# Autodesk Inventor assembly: x_motor
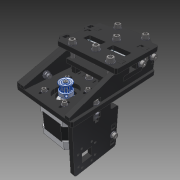
[picture p0: Inventor's stored thumbnail of the model, 180x180]
Saved by Autodesk Inventor 2014 (Build 180170000, 170)
## iProperties
Created: 2014-01-10
Part Number: x_motor
Document SubType Name: Assembly
Designer: buben
Author: buben
## Documents named in this file (23)
- C:\Users\buben\Documents\GitHub\bacon\inventor files\assemblies\x_motor.iam
- C:\Users\buben\Documents\GitHub\bacon\inventor files\printer parts\x_motor_back.ipt
- C:\Users\buben\Documents\GitHub\bacon\inventor files\printer parts\x_motor_wall_lower.ipt
- C:\Users\buben\Documents\GitHub\bacon\inventor files\printer parts\x_motor_wall_upper.ipt
- C:\Users\buben\Documents\GitHub\bacon\inventor files\printer parts\x_motor_middle.ipt
- C:\Users\buben\Documents\GitHub\bacon\inventor files\printer parts\x_motor_smooth_rod_spacer.ipt
- C:\Users\buben\Documents\GitHub\bacon\inventor files\3rd party components\linear_bearing_8\Imported Components\LU8MM\LU8MM.iam
- C:\Users\buben\Documents\GitHub\bacon\inventor files\printer parts\x_motor_top.ipt
- C:\Users\buben\Documents\GitHub\bacon\inventor files\printer parts\x_motor_upper_nut_stop.ipt
- C:\Users\buben\Documents\GitHub\bacon\inventor files\printer parts\x_motor_lower_nut_stop.ipt
- C:\Users\buben\Documents\GitHub\bacon\inventor files\utils\washer_m5.ipt
- C:\Users\buben\Documents\Inventor\Content Center Files\R2014\en-US\ISO 4762(2)\ISO 4762 - M5 x 45ISO.ipt
- C:\Users\buben\Documents\Inventor\Content Center Files\R2014\en-US\ISO 7040\ISO 7040 - M5.ipt
- C:\Users\buben\Documents\GitHub\bacon\inventor files\utils\washer_m4.ipt
- C:\Users\buben\Documents\Inventor\Content Center Files\R2014\en-US\ISO 4762(2)\ISO 4762 - M4 x 20ISO.ipt
- C:\Users\buben\Documents\Inventor\Content Center Files\R2014\en-US\ISO 7040\ISO 7040 - M4.ipt
- C:\Users\buben\Documents\GitHub\bacon\inventor files\printer parts\x_motor_cable_mount.ipt
- C:\Users\buben\Documents\GitHub\bacon\inventor files\printer parts\x_motor_cable_mount_brace.ipt
- C:\Users\buben\Documents\Inventor\Content Center Files\R2014\en-US\CSN EN 24032\ISO 4032 - M5CSN EN.ipt
- C:\Users\buben\Documents\GitHub\bacon\inventor files\printer parts\motor_spacer.ipt
- C:\Users\buben\Documents\GitHub\bacon\inventor files\3rd party components\nema_17_stepper\Imported Components\NEMA 17 with T5 Pulley\NEMA 17 with T5 Pulley.iam
- C:\Users\buben\Documents\GitHub\bacon\inventor files\utils\washer_m3.ipt
- C:\Users\buben\Documents\Inventor\Content Center Files\R2014\en-US\ISO 4762(2)\ISO 4762 - M3 x 16ISO.ipt
## Components (73 placed, 22 different names)
1. x_motor_back:1 — Mate:1, Flush:1, Mate:2, Mate:4, Mate:5, Mate:6, Mate:7, Mate:8, Mate:9, Mate:12, Mate:13, Mate:14, Mate:15, Mate:16, Mate:17, Mate:33, Mate:34, Mate:47, Mate:48, Mate:49, Mate:50, Mate:51, Mate:52, Mate:101, Mate:102, Mate:103, Mate:104, Mate:105, Mate:106, Mate:107, Mate:109, Mate:131, Tangent:1, Tangent:2, Mate:135, Mate:136, Mate:137, Mate:138
2. x_motor_wall_lower:1 — Mate:7, Mate:8, Mate:9, Mate:27, Mate:28, Mate:30, Mate:31, Mate:80, Mate:81, Mate:82, Mate:83, Mate:125, Mate:126
3. x_motor_wall_upper:1 — Mate:4, Mate:5, Mate:6, Mate:10, Mate:11, Mate:18, Mate:32, Mate:77, Mate:128, Mate:129
4. x_motor_middle:1 — Mate:10, Mate:11, Mate:18, Mate:19, Mate:20, Mate:21, Mate:22, Mate:23, Mate:24, Mate:29
5. x_motor_smooth_rod_spacer:1 — Mate:12, Mate:13, Mate:14
6. x_motor_smooth_rod_spacer:2 — Mate:15, Mate:16, Mate:17
7. LU8MM:1 [sub-assembly] — Mate:21, Mate:22, Mate:24
8. LU8MM:2 [sub-assembly] — Mate:19, Mate:20, Mate:23, Mate:25, Mate:26
9. x_motor_top:1 — Mate:25, Mate:26, Mate:27, Mate:28, Mate:35, Mate:36, Mate:37, Mate:38, Mate:39, Mate:40, Mate:41, Mate:42, Mate:43, Mate:44, Mate:45, Mate:46
10. x_motor_upper_nut_stop:1 — Mate:32, Mate:33, Mate:34, Mate:71, Mate:76, Mate:130
11. x_motor_lower_nut_stop:1 — Mate:29, Mate:30, Mate:31, Mate:84, Mate:85, Mate:127
12. CSN 02 1702 B B 5,3:1 — Mate:40, Mate:44, Insert:5
13. CSN 02 1702 B B 5,3:2 — Mate:38, Mate:42, Insert:2
14. CSN 02 1702 B B 5,3:3 — Mate:39, Mate:45, Insert:6
15. CSN 02 1702 B B 5,3:4 — Mate:37, Mate:46, Insert:3
16. CSN 02 1702 B B 5,3:5 — Mate:36, Mate:41, Insert:1
17. CSN 02 1702 B B 5,3:6 — Mate:35, Mate:43, Insert:4
18. CSN 02 1702 B B 5,3:7 — Mate:48, Mate:57, Mate:61
19. CSN 02 1702 B B 5,3:8 — Mate:51, Mate:54, Mate:63
20. CSN 02 1702 B B 5,3:9 — Mate:47, Mate:53, Mate:69
21. CSN 02 1702 B B 5,3:10 — Mate:49, Mate:56, Mate:65
22. CSN 02 1702 B B 5,3:11 — Mate:50, Mate:55, Mate:67
23. CSN 02 1702 B B 5,3:12 — Mate:52, Mate:58, Mate:59
24. ISO 4762 M5 x 45:1 — Insert:1, Mate:53, Mate:70
25. ISO 4762 M5 x 45:2 — Insert:2, Mate:54, Mate:64
26. ISO 4762 M5 x 45:3 — Insert:3, Mate:58, Mate:60
27. ISO 4762 M5 x 45:4 — Insert:4, Mate:56, Mate:66
28. ISO 4762 M5 x 45:5 — Insert:5, Mate:55, Mate:68
29. ISO 4762 M5 x 45:6 — Insert:6, Mate:57, Mate:62
30. DIN EN ISO 7040 M5:1 — Mate:69, Mate:70
31. DIN EN ISO 7040 M5:2 — Mate:67, Mate:68
32. DIN EN ISO 7040 M5:3 — Mate:65, Mate:66
33. DIN EN ISO 7040 M5:4 — Mate:63, Mate:64
34. DIN EN ISO 7040 M5:5 — Mate:61, Mate:62
35. DIN EN ISO 7040 M5:6 — Mate:59, Mate:60
36. CSN 02 1702 B B 4,3:2 — Mate:77, Mate:90, Mate:91
37. CSN 02 1702 B B 4,3:4 — Mate:71, Mate:76, Insert:7
38. CSN 02 1702 B B 4,3:7 — Mate:84, Mate:88, Mate:97
39. CSN 02 1702 B B 4,3:8 — Mate:85, Mate:89, Mate:99
40. CSN 02 1702 B B 4,3:9 — Mate:81, Mate:83, Insert:11
41. CSN 02 1702 B B 4,3:10 — Mate:80, Mate:82, Insert:10
42. ISO 4762 M4 x 20:1 — Insert:7, Mate:90, Mate:92
43. ISO 4762 M4 x 20:4 — Insert:10, Mate:89, Mate:100
44. ISO 4762 M4 x 20:5 — Insert:11, Mate:88, Mate:98
45. DIN EN ISO 7040 M4:3 — Mate:97, Mate:98
46. DIN EN ISO 7040 M4:4 — Mate:99, Mate:100
47. DIN EN ISO 7040 M4:5 — Mate:91, Mate:92
48. CSN 02 1702 B B 4,3:11 — Mate:101, Mate:102, Insert:12
49. CSN 02 1702 B B 4,3:12 — Mate:103, Mate:104, Insert:13
50. ISO 4762 M4 x 20:6 — Insert:12, Mate:118, Mate:124
51. ISO 4762 M4 x 20:7 — Insert:13, Mate:116, Mate:122
52. CSN 02 1702 B B 4,3:13 — Mate:115, Mate:116, Mate:121
53. CSN 02 1702 B B 4,3:14 — Mate:117, Mate:118, Mate:123
54. x_motor_cable_mount:1 — Mate:105, Mate:106, Mate:107, Mate:108, Mate:110, Mate:111, Mate:112, Mate:117
55. x_motor_cable_mount_brace:1 — Mate:108, Mate:109, Mate:110, Mate:113, Mate:115
56. CSN 02 1702 B B 4,3:15 — Mate:113, Mate:114, Mate:119
57. CSN 02 1702 B B 4,3:16 — Mate:111, Mate:112, Insert:14
58. ISO 4762 M4 x 20:8 — Insert:14, Mate:114, Mate:120
59. DIN EN ISO 7040 M4:6 — Mate:123, Mate:124
60. DIN EN ISO 7040 M4:7 — Mate:121, Mate:122
61. DIN EN ISO 7040 M4:8 — Mate:119, Mate:120
62. CSN EN 24032 M5:1 — Mate:128, Mate:129, Mate:130
63. CSN EN 24032 M5:2 — Mate:125, Mate:126, Mate:127
64. motor_spacer:1 — Mate:131, Tangent:1, Tangent:2, Mate:132, Mate:133, Mate:134, Mate:139, Mate:140, Mate:141, Mate:142
65. NEMA 17 with T5 Pulley:1 [sub-assembly] — Mate:132, Mate:133, Mate:134
66. CSN 02 1702 B B 3,2:1 — Mate:135, Insert:16
67. CSN 02 1702 B B 3,2:2 — Mate:136, Insert:15
68. CSN 02 1702 B B 3,2:3 — Mate:137, Insert:17
69. CSN 02 1702 B B 3,2:4 — Mate:138, Insert:18
70. ISO 4762 M3 x 16:1 — Insert:16, Mate:141
71. ISO 4762 M3 x 16:2 — Insert:15, Mate:139
72. ISO 4762 M3 x 16:3 — Insert:17, Mate:142
73. ISO 4762 M3 x 16:4 — Insert:18, Mate:140
## Relationships (148: Mate 129, Insert 16, Tangent 2, Flush 1)
- Mate:1: x_motor_back:1
- Flush:1: x_motor_back:1
- Mate:2: x_motor_back:1
- Mate:4: x_motor_back:1 ↔ x_motor_wall_upper:1
- Mate:5: x_motor_back:1 ↔ x_motor_wall_upper:1
- Mate:6: x_motor_back:1 ↔ x_motor_wall_upper:1
- Mate:7: x_motor_back:1 ↔ x_motor_wall_lower:1
- Mate:8: x_motor_back:1 ↔ x_motor_wall_lower:1
- Mate:9: x_motor_back:1 ↔ x_motor_wall_lower:1
- Mate:10: x_motor_wall_upper:1 ↔ x_motor_middle:1
- Mate:11: x_motor_wall_upper:1 ↔ x_motor_middle:1
- Mate:12: x_motor_back:1 ↔ x_motor_smooth_rod_spacer:1
- Mate:13: x_motor_back:1 ↔ x_motor_smooth_rod_spacer:1
- Mate:14: x_motor_back:1 ↔ x_motor_smooth_rod_spacer:1
- Mate:15: x_motor_back:1 ↔ x_motor_smooth_rod_spacer:2
- Mate:16: x_motor_back:1 ↔ x_motor_smooth_rod_spacer:2
- Mate:17: x_motor_back:1 ↔ x_motor_smooth_rod_spacer:2
- Mate:18: x_motor_wall_upper:1 ↔ x_motor_middle:1
- Mate:19 (7.5 mm): x_motor_middle:1 ↔ LU8MM:2
- Mate:20 (7.5 mm): x_motor_middle:1 ↔ LU8MM:2
- Mate:21 (7.5 mm): x_motor_middle:1 ↔ LU8MM:1
- Mate:22 (7.5 mm): x_motor_middle:1 ↔ LU8MM:1
- Mate:23 (0.5 mm): x_motor_middle:1 ↔ LU8MM:2
- Mate:24 (0.5 mm): x_motor_middle:1 ↔ LU8MM:1
- Mate:25 (7.5 mm): LU8MM:2 ↔ x_motor_top:1
- Mate:26 (7.5 mm): LU8MM:2 ↔ x_motor_top:1
- Mate:27: x_motor_wall_lower:1 ↔ x_motor_top:1
- Mate:28: x_motor_wall_lower:1 ↔ x_motor_top:1
- Mate:29: x_motor_middle:1 ↔ x_motor_lower_nut_stop:1
- Mate:30: x_motor_wall_lower:1 ↔ x_motor_lower_nut_stop:1
- Mate:31: x_motor_wall_lower:1 ↔ x_motor_lower_nut_stop:1
- Mate:32: x_motor_wall_upper:1 ↔ x_motor_upper_nut_stop:1
- Mate:33: x_motor_back:1 ↔ x_motor_upper_nut_stop:1
- Mate:34: x_motor_back:1 ↔ x_motor_upper_nut_stop:1
- Mate:35: x_motor_top:1 ↔ CSN 02 1702 B B 5,3:6
- Mate:36: x_motor_top:1 ↔ CSN 02 1702 B B 5,3:5
- Mate:37: x_motor_top:1 ↔ CSN 02 1702 B B 5,3:4
- Mate:38: x_motor_top:1 ↔ CSN 02 1702 B B 5,3:2
- Mate:39: x_motor_top:1 ↔ CSN 02 1702 B B 5,3:3
- Mate:40: x_motor_top:1 ↔ CSN 02 1702 B B 5,3:1
- Mate:41: x_motor_top:1 ↔ CSN 02 1702 B B 5,3:5
- Mate:42: x_motor_top:1 ↔ CSN 02 1702 B B 5,3:2
- Mate:43: x_motor_top:1 ↔ CSN 02 1702 B B 5,3:6
- Mate:44: x_motor_top:1 ↔ CSN 02 1702 B B 5,3:1
- Mate:45: x_motor_top:1 ↔ CSN 02 1702 B B 5,3:3
- Mate:46: x_motor_top:1 ↔ CSN 02 1702 B B 5,3:4
- Mate:47: x_motor_back:1 ↔ CSN 02 1702 B B 5,3:9
- Mate:48: x_motor_back:1 ↔ CSN 02 1702 B B 5,3:7
- Mate:49: x_motor_back:1 ↔ CSN 02 1702 B B 5,3:10
- Mate:50: x_motor_back:1 ↔ CSN 02 1702 B B 5,3:11
- Mate:51: x_motor_back:1 ↔ CSN 02 1702 B B 5,3:8
- Mate:52: x_motor_back:1 ↔ CSN 02 1702 B B 5,3:12
- Insert:1: CSN 02 1702 B B 5,3:5 ↔ ISO 4762 M5 x 45:1
- Insert:2: CSN 02 1702 B B 5,3:2 ↔ ISO 4762 M5 x 45:2
- Insert:3: CSN 02 1702 B B 5,3:4 ↔ ISO 4762 M5 x 45:3
- Insert:4: CSN 02 1702 B B 5,3:6 ↔ ISO 4762 M5 x 45:4
- Insert:5: CSN 02 1702 B B 5,3:1 ↔ ISO 4762 M5 x 45:5
- Insert:6: CSN 02 1702 B B 5,3:3 ↔ ISO 4762 M5 x 45:6
- Mate:53: CSN 02 1702 B B 5,3:9 ↔ ISO 4762 M5 x 45:1
- Mate:54: CSN 02 1702 B B 5,3:8 ↔ ISO 4762 M5 x 45:2
- Mate:55: CSN 02 1702 B B 5,3:11 ↔ ISO 4762 M5 x 45:5
- Mate:56: CSN 02 1702 B B 5,3:10 ↔ ISO 4762 M5 x 45:4
- Mate:57: CSN 02 1702 B B 5,3:7 ↔ ISO 4762 M5 x 45:6
- Mate:58: CSN 02 1702 B B 5,3:12 ↔ ISO 4762 M5 x 45:3
- Mate:59: CSN 02 1702 B B 5,3:12 ↔ DIN EN ISO 7040 M5:6
- Mate:60: ISO 4762 M5 x 45:3 ↔ DIN EN ISO 7040 M5:6
- Mate:61: CSN 02 1702 B B 5,3:7 ↔ DIN EN ISO 7040 M5:5
- Mate:62: ISO 4762 M5 x 45:6 ↔ DIN EN ISO 7040 M5:5
- Mate:63: CSN 02 1702 B B 5,3:8 ↔ DIN EN ISO 7040 M5:4
- Mate:64: ISO 4762 M5 x 45:2 ↔ DIN EN ISO 7040 M5:4
- Mate:65: CSN 02 1702 B B 5,3:10 ↔ DIN EN ISO 7040 M5:3
- Mate:66: ISO 4762 M5 x 45:4 ↔ DIN EN ISO 7040 M5:3
- Mate:67: CSN 02 1702 B B 5,3:11 ↔ DIN EN ISO 7040 M5:2
- Mate:68: ISO 4762 M5 x 45:5 ↔ DIN EN ISO 7040 M5:2
- Mate:69: CSN 02 1702 B B 5,3:9 ↔ DIN EN ISO 7040 M5:1
- Mate:70: ISO 4762 M5 x 45:1 ↔ DIN EN ISO 7040 M5:1
- Mate:71: x_motor_upper_nut_stop:1 ↔ CSN 02 1702 B B 4,3:4
- Mate:76: x_motor_upper_nut_stop:1 ↔ CSN 02 1702 B B 4,3:4
- Mate:77: x_motor_wall_upper:1 ↔ CSN 02 1702 B B 4,3:2
- Mate:80: x_motor_wall_lower:1 ↔ CSN 02 1702 B B 4,3:10
- Mate:81: x_motor_wall_lower:1 ↔ CSN 02 1702 B B 4,3:9
- Mate:82: x_motor_wall_lower:1 ↔ CSN 02 1702 B B 4,3:10
- Mate:83: x_motor_wall_lower:1 ↔ CSN 02 1702 B B 4,3:9
- Mate:84: x_motor_lower_nut_stop:1 ↔ CSN 02 1702 B B 4,3:7
- Mate:85: x_motor_lower_nut_stop:1 ↔ CSN 02 1702 B B 4,3:8
- Insert:7: CSN 02 1702 B B 4,3:4 ↔ ISO 4762 M4 x 20:1
- Insert:10: CSN 02 1702 B B 4,3:10 ↔ ISO 4762 M4 x 20:4
- Insert:11: CSN 02 1702 B B 4,3:9 ↔ ISO 4762 M4 x 20:5
- Mate:88: CSN 02 1702 B B 4,3:7 ↔ ISO 4762 M4 x 20:5
- Mate:89: CSN 02 1702 B B 4,3:8 ↔ ISO 4762 M4 x 20:4
- Mate:90: CSN 02 1702 B B 4,3:2 ↔ ISO 4762 M4 x 20:1
- Mate:91: CSN 02 1702 B B 4,3:2 ↔ DIN EN ISO 7040 M4:5
- Mate:92: ISO 4762 M4 x 20:1 ↔ DIN EN ISO 7040 M4:5
- Mate:97: CSN 02 1702 B B 4,3:7 ↔ DIN EN ISO 7040 M4:3
- Mate:98: ISO 4762 M4 x 20:5 ↔ DIN EN ISO 7040 M4:3
- Mate:99: CSN 02 1702 B B 4,3:8 ↔ DIN EN ISO 7040 M4:4
- Mate:100: ISO 4762 M4 x 20:4 ↔ DIN EN ISO 7040 M4:4
- Mate:101: x_motor_back:1 ↔ CSN 02 1702 B B 4,3:11
- Mate:102: x_motor_back:1 ↔ CSN 02 1702 B B 4,3:11
- Insert:12: CSN 02 1702 B B 4,3:11 ↔ ISO 4762 M4 x 20:6
- Mate:103: x_motor_back:1 ↔ CSN 02 1702 B B 4,3:12
- Mate:104: x_motor_back:1 ↔ CSN 02 1702 B B 4,3:12
- Insert:13: CSN 02 1702 B B 4,3:12 ↔ ISO 4762 M4 x 20:7
- Mate:105: x_motor_back:1 ↔ x_motor_cable_mount:1
- Mate:106: x_motor_back:1 ↔ x_motor_cable_mount:1
- Mate:107: x_motor_back:1 ↔ x_motor_cable_mount:1
- Mate:108: x_motor_cable_mount:1 ↔ x_motor_cable_mount_brace:1
- Mate:109: x_motor_back:1 ↔ x_motor_cable_mount_brace:1
- Mate:110: x_motor_cable_mount:1 ↔ x_motor_cable_mount_brace:1
- Mate:111: x_motor_cable_mount:1 ↔ CSN 02 1702 B B 4,3:16
- Mate:112: x_motor_cable_mount:1 ↔ CSN 02 1702 B B 4,3:16
- Insert:14: CSN 02 1702 B B 4,3:16 ↔ ISO 4762 M4 x 20:8
- Mate:113: x_motor_cable_mount_brace:1 ↔ CSN 02 1702 B B 4,3:15
- Mate:114: CSN 02 1702 B B 4,3:15 ↔ ISO 4762 M4 x 20:8
- Mate:115: CSN 02 1702 B B 4,3:13 ↔ x_motor_cable_mount_brace:1
- Mate:116: ISO 4762 M4 x 20:7 ↔ CSN 02 1702 B B 4,3:13
- Mate:117: CSN 02 1702 B B 4,3:14 ↔ x_motor_cable_mount:1
- Mate:118: ISO 4762 M4 x 20:6 ↔ CSN 02 1702 B B 4,3:14
- Mate:119: CSN 02 1702 B B 4,3:15 ↔ DIN EN ISO 7040 M4:8
- Mate:120: ISO 4762 M4 x 20:8 ↔ DIN EN ISO 7040 M4:8
- Mate:121: CSN 02 1702 B B 4,3:13 ↔ DIN EN ISO 7040 M4:7
- Mate:122: ISO 4762 M4 x 20:7 ↔ DIN EN ISO 7040 M4:7
- Mate:123: CSN 02 1702 B B 4,3:14 ↔ DIN EN ISO 7040 M4:6
- Mate:124: ISO 4762 M4 x 20:6 ↔ DIN EN ISO 7040 M4:6
- Mate:125: x_motor_wall_lower:1 ↔ CSN EN 24032 M5:2
- Mate:126: x_motor_wall_lower:1 ↔ CSN EN 24032 M5:2
- Mate:127: x_motor_lower_nut_stop:1 ↔ CSN EN 24032 M5:2
- Mate:128: x_motor_wall_upper:1 ↔ CSN EN 24032 M5:1
- Mate:129: x_motor_wall_upper:1 ↔ CSN EN 24032 M5:1
- Mate:130: x_motor_upper_nut_stop:1 ↔ CSN EN 24032 M5:1
- Mate:131: x_motor_back:1 ↔ motor_spacer:1
- Tangent:1: x_motor_back:1 ↔ motor_spacer:1
- Tangent:2: x_motor_back:1 ↔ motor_spacer:1
- Mate:132: motor_spacer:1 ↔ NEMA 17 with T5 Pulley:1
- Mate:133: motor_spacer:1 ↔ NEMA 17 with T5 Pulley:1
- Mate:134: motor_spacer:1 ↔ NEMA 17 with T5 Pulley:1
- Mate:135: x_motor_back:1 ↔ CSN 02 1702 B B 3,2:1
- Mate:136: x_motor_back:1 ↔ CSN 02 1702 B B 3,2:2
- Mate:137: x_motor_back:1 ↔ CSN 02 1702 B B 3,2:3
- Mate:138: x_motor_back:1 ↔ CSN 02 1702 B B 3,2:4
- Insert:15: CSN 02 1702 B B 3,2:2 ↔ ISO 4762 M3 x 16:2
- Insert:16: CSN 02 1702 B B 3,2:1 ↔ ISO 4762 M3 x 16:1
- Insert:17: CSN 02 1702 B B 3,2:3 ↔ ISO 4762 M3 x 16:3
- Insert:18: CSN 02 1702 B B 3,2:4 ↔ ISO 4762 M3 x 16:4
- Mate:139: motor_spacer:1 ↔ ISO 4762 M3 x 16:2
- Mate:140: motor_spacer:1 ↔ ISO 4762 M3 x 16:4
- Mate:141: motor_spacer:1 ↔ ISO 4762 M3 x 16:1
- Mate:142: motor_spacer:1 ↔ ISO 4762 M3 x 16:3
